# Autodesk Inventor assembly: Assembly PCB_1DOF
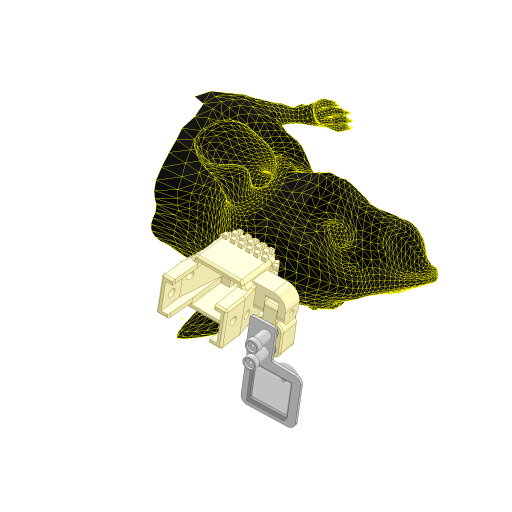
[picture p0: Inventor's stored thumbnail of the model, 512x512]
Saved by Autodesk Inventor 2023 (Build 270158000, 158)
## iProperties
Created: 2024-02-19
Part Number: Assembly PCB_1DOF
Document SubType Name: Assembly
Designer: ferrerx
Author: ferrerx
## Documents named in this file (8)
- C:\Users\ferrerx\Desktop\Projects\Iacaruso Lab\MSTP00347 - Neuropixels eye tracking\Assembly PCB_1DOF.iam
- C:\Users\ferrerx\Desktop\Projects\Iacaruso Lab\MSTP00347 - Neuropixels eye tracking\head.ipt
- C:\Users\ferrerx\Desktop\Projects\Iacaruso Lab\MSTP00347 - Neuropixels eye tracking\SIL connector.ipt
- C:\Users\ferrerx\Desktop\Projects\Iacaruso Lab\MSTP00347 - Neuropixels eye tracking\SIL connector cut.ipt
- C:\Users\ferrerx\Desktop\Projects\Iacaruso Lab\MSTP00347 - Neuropixels eye tracking\PCB_arm.ipt
- C:\Users\ferrerx\Desktop\Projects\Iacaruso Lab\MSTP00347 - Neuropixels eye tracking\Camera.ipt
- C:\Users\ferrerx\Desktop\Projects\Iacaruso Lab\MSTP00347 - Neuropixels eye tracking\Camera_holder_PCB_1DOF.ipt
- C:\Users\ferrerx\Desktop\Projects\Iacaruso Lab\MSTP00347 - Neuropixels eye tracking\NP2_Docking_PCB_1DOF.ipt
## Components (9 placed, 7 different names)
1. head:1
2. SIL connector:1 — Mate:13, Flush:3, Flush:4, Mate:16
3. SIL connector:2 — Mate:14, Flush:4, Mate:15, Mate:21
4. SIL connector cut:1 — Mate:15, Mate:19, Flush:6, Mate:21
5. SIL connector cut:2 — Mate:16, Mate:20, Flush:5
6. PCB_arm:1 — Mate:8, Mate:9, Mate:10, Mate:13, Flush:3, Mate:14
7. Camera:1 — Mate:8, Mate:9, Mate:10
8. Camera_holder_PCB_1DOF:1 — Mate:17, Mate:18, Mate:19, Mate:20, Flush:5, Flush:6
9. NP2_Docking_PCB_1DOF:1 — Mate:17, Mate:18
## Relationships (16: Mate 12, Flush 4)
- Mate:8: PCB_arm:1 ↔ Camera:1
- Mate:9 (0.15 mm): PCB_arm:1 ↔ Camera:1
- Mate:10 (0.15 mm): PCB_arm:1 ↔ Camera:1
- Mate:13: SIL connector:1 ↔ PCB_arm:1
- Flush:3 (-3 mm): SIL connector:1 ↔ PCB_arm:1
- Mate:14: SIL connector:2 ↔ PCB_arm:1
- Flush:4: SIL connector:1 ↔ SIL connector:2
- Mate:15: SIL connector:2 ↔ SIL connector cut:1
- Mate:16: SIL connector:1 ↔ SIL connector cut:2
- Mate:17: Camera_holder_PCB_1DOF:1 ↔ NP2_Docking_PCB_1DOF:1
- Mate:18 (0.1 mm): Camera_holder_PCB_1DOF:1 ↔ NP2_Docking_PCB_1DOF:1
- Mate:19: SIL connector cut:1 ↔ Camera_holder_PCB_1DOF:1
- Mate:20: SIL connector cut:2 ↔ Camera_holder_PCB_1DOF:1
- Flush:5: SIL connector cut:2 ↔ Camera_holder_PCB_1DOF:1
- Flush:6: SIL connector cut:1 ↔ Camera_holder_PCB_1DOF:1
- Mate:21: SIL connector:2 ↔ SIL connector cut:1
